# Autodesk Inventor assembly: Estructura
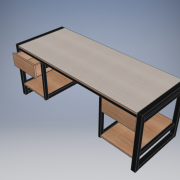
[picture p0: Inventor's stored thumbnail of the model, 180x180]
Saved by Autodesk Inventor 2016 (Build 200138000, 138)
## iProperties
Created: 2018-06-24
Part Number: Estructura
Document SubType Name: Assembly
Designer: damia
_SolveAssemblyDoc: Frame Generator Solve Assembly
_Version: 15.0.0
Author: damia
## Documents named in this file (7)
- C:\Users\damia\Documents\Inventor\Escritorio_Sebastian\Estructura.iam
- C:\Users\damia\Documents\Inventor\Escritorio_Sebastian\Esqueleto.ipt
- C:\Users\damia\Documents\Inventor\Escritorio_Sebastian\Estructura\Frame\Frame0002.iam
- C:\Users\damia\Documents\Inventor\Escritorio_Sebastian\Part42.ipt
- C:\Users\damia\Documents\Inventor\Escritorio_Sebastian\tablero_granded.ipt
- C:\Users\damia\Documents\Inventor\Escritorio_Sebastian\FrenteGrande.ipt
- C:\Users\damia\Documents\Inventor\Escritorio_Sebastian\FrenteChico.ipt
## Components (8 placed, 6 different names)
1. Esqueleto:1 — Mate:1, Mate:2
2. Frame0002:1 [sub-assembly] — Mate:6, Mate:7, Mate:8, Mate:9, Mate:10, Flush:7, Flush:8, Mate:11, Mate:12, Flush:9, Flush:10
3. tablero_granded:1 — Mate:10
4. VidrioGrande:1
5. FrenteGrande:1 — Mate:7, Mate:8
6. FrenteGrande:2 — Mate:6, Mate:9
7. FrenteChico:1 — Flush:7, Mate:12, Flush:9
8. FrenteChico:2 — Flush:8, Mate:11, Flush:10
## Relationships (17: Mate 10, Flush 7)
- Mate:1: Esqueleto:1
- Mate:2: Esqueleto:1
- [Flush]: tablero_granded:1 ↔ VidrioGrande:1
- [Flush]: tablero_granded:1 ↔ VidrioGrande:1
- [Mate]: Frame0002:1 ↔ tablero_granded:1
- [Flush]: Frame0002:1 ↔ tablero_granded:1
- Mate:6 (5 mm): Frame0002:1 ↔ FrenteGrande:2
- Mate:7: Frame0002:1 ↔ FrenteGrande:1
- Mate:8 (5 mm): Frame0002:1 ↔ FrenteGrande:1
- Mate:9 (5 mm): Frame0002:1 ↔ FrenteGrande:2
- Mate:10: Frame0002:1 ↔ tablero_granded:1
- Flush:7: Frame0002:1 ↔ FrenteChico:1
- Flush:8: Frame0002:1 ↔ FrenteChico:2
- Mate:11: Frame0002:1 ↔ FrenteChico:2
- Mate:12: Frame0002:1 ↔ FrenteChico:1
- Flush:9 (15 mm): Frame0002:1 ↔ FrenteChico:1
- Flush:10 (-15 mm): Frame0002:1 ↔ FrenteChico:2
## Named parameters: d16_d6 = 0 mm
